# Autodesk Inventor assembly: magplate_blank
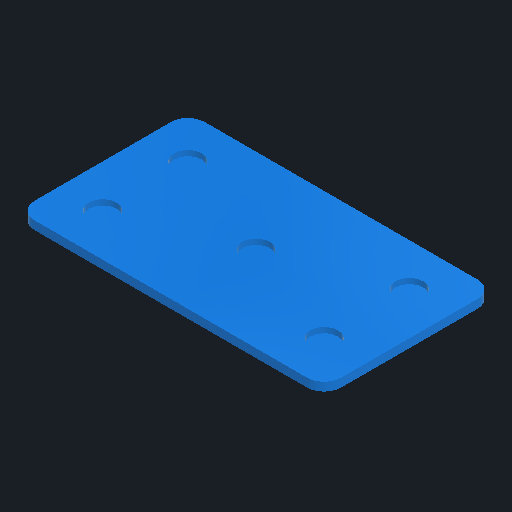
[picture p0: Inventor's stored thumbnail of the model, 512x512]
Saved by Autodesk Inventor 2025 (Build 290162000, 162)
## iProperties
Created: 2024-06-22
Part Number: magplate_blank
Document SubType Name: Assembly
Designer: AdminForWorker
Title: magplate_blank v6
Author: AdminForWorker
## Documents named in this file (5)
- D:\VEX\High Stakes\CAD\ROBOPROS-CAD-Inventor\Miscellaneous\Magplates\Plate\!Plate.iam
- D:\VEX\High Stakes\CAD\ROBOPROS-CAD-Inventor\Miscellaneous\Magplates\Plate\Text.ipt
- D:\VEX\High Stakes\CAD\ROBOPROS-CAD-Inventor\Miscellaneous\Magplates\Plate\Logo.ipt
- D:\VEX\High Stakes\CAD\ROBOPROS-CAD-Inventor\Miscellaneous\Magplates\Plate\Plate.ipt
- D:\VEX\High Stakes\CAD\ROBOPROS-CAD-Inventor\Miscellaneous\Magplates\Plate\Rim.ipt
## Components (4 placed, 3 different names)
1. Text
2. Rim
3. Plate — Flush:1
4. Rim:1 — Flush:1
## Relationships (1: Flush 1)
- Flush:1: Plate ↔ Rim:1
